# Autodesk Inventor assembly: MECANISMO DE COMPACTADO
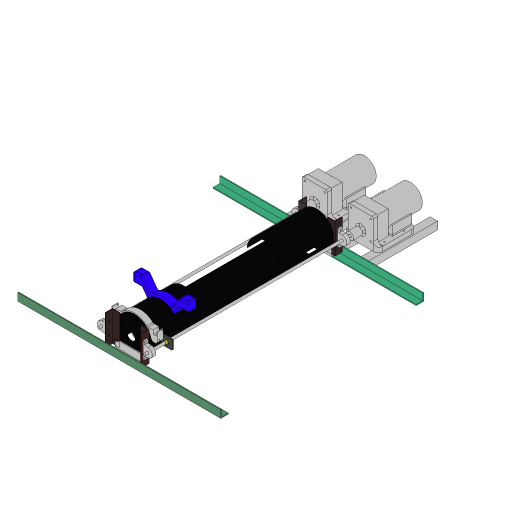
[picture p0: Inventor's stored thumbnail of the model, 512x512]
Saved by Autodesk Inventor 2024 (Build 280153000, 153)
## iProperties
Created: 2024-05-26
Part Number: MECANISMO DE COMPACTADO
Document SubType Name: Assembly
Designer: Jhuliams
Author: Jhuliams
## Documents named in this file (14)
- C:\Users\Jhuliams\Documents\GitHub\RECICLADOR_MODELO_3D\MECANISMO DE COMPACTADO\MECANISMO DE COMPACTADO.iam
- C:\Users\Jhuliams\Documents\GitHub\RECICLADOR_MODELO_3D\MECANISMO DE COMPACTADO\GUIA_DE_OBJETO.ipt
- C:\Users\Jhuliams\Documents\GitHub\RECICLADOR_MODELO_3D\MECANISMO DE COMPACTADO\TAPA QUE DESPLAZA CON TORNILLOS.ipt
- C:\Users\Jhuliams\Documents\GitHub\RECICLADOR_MODELO_3D\MECANISMO DE COMPACTADO\TUERCA DE HUSILLO.ipt
- C:\Users\Jhuliams\Documents\GitHub\RECICLADOR_MODELO_3D\MECANISMO DE COMPACTADO\TORNILLO DEPOTENCIA.ipt
- C:\Users\Jhuliams\Documents\GitHub\RECICLADOR_MODELO_3D\MECANISMO DE COMPACTADO\ACOPLE HELICOIDAL.ipt
- C:\Users\Jhuliams\Documents\GitHub\RECICLADOR_MODELO_3D\MECANISMO DE COMPACTADO\MOTOR DC.ipt
- C:\Users\Jhuliams\Documents\GitHub\RECICLADOR_MODELO_3D\MECANISMO DE COMPACTADO\RODAMIENTO DE TORNILLO.ipt
- C:\Users\Jhuliams\Documents\GitHub\RECICLADOR_MODELO_3D\MECANISMO DE COMPACTADO\SOPORTE DEL MOTOR.ipt
- C:\Users\Jhuliams\Documents\GitHub\RECICLADOR_MODELO_3D\MECANISMO DE COMPACTADO\SOPORTE LATERAL DE GUIA CILINDRICA.ipt
- C:\Users\Jhuliams\Documents\GitHub\RECICLADOR_MODELO_3D\MECANISMO DE COMPACTADO\PERFIL_SOPORTE DE CILINDRO.ipt
- C:\Users\Jhuliams\Documents\GitHub\RECICLADOR_MODELO_3D\MECANISMO DE COMPACTADO\PERFIL_SOPORTE DEL MOTOR.ipt
- C:\Users\Jhuliams\Documents\GitHub\RECICLADOR_MODELO_3D\MECANISMO DE COMPACTADO\SOPORTE DE SENSOR INFRARROJO.ipt
- C:\Users\Jhuliams\Documents\GitHub\RECICLADOR_MODELO_3D\MECANISMO DE COMPACTADO\SOPORTE FIN DE CARRERA.ipt
## Components (30 placed, 13 different names)
1. PERFIL_SOPORTE DE CILINDRO:1 — Mate:2, Flush:1, Mate:4, Flush:3, Mate:49
2. SOPORTE LATERAL DE GUIA CILINDRICA:5 — Mate:1, Mate:3, Mate:5, Flush:2, Mate:6, Mate:8
3. SOPORTE LATERAL DE GUIA CILINDRICA:6 — Mate:2, Mate:4, Mate:5, Flush:2, Mate:7
4. PERFIL_SOPORTE DE CILINDRO:3 — Mate:1, Flush:1, Mate:3, Flush:3, Flush:4, Flush:17
5. GUIA_DE_OBJETO:1 — Mate:6, Mate:7, Flush:4, Mate:8, Mate:9, Mate:10, Mate:34, Mate:35, Mate:65, Mate:66
6. TAPA QUE DESPLAZA CON TORNILLOS:1 — Mate:9, Mate:10, Mate:11, Mate:12, Mate:13, Mate:14, Mate:15
7. TUERCA DE HUSILLO:1 — Mate:12, Mate:13, Flush:5, Mate:15, Mate:16
8. TUERCA DE HUSILLO:2 — Mate:11, Mate:14, Flush:5, Mate:17
9. TORNILLO DEPOTENCIA:1 — Mate:16, Flush:6, Mate:30, Mate:33, Mate:36, Mate:37, Mate:39
10. TORNILLO DEPOTENCIA:2 — Mate:17, Flush:6, Mate:31, Mate:32, Mate:38, Mate:40
11. SOPORTE LATERAL DE GUIA CILINDRICA:7 — Mate:20, Mate:21, Mate:26, Flush:7, Flush:8, Mate:35, Flush:17
12. SOPORTE LATERAL DE GUIA CILINDRICA:8 — Mate:22, Mate:23, Mate:27, Flush:7, Flush:8
13. SOPORTE LATERAL DE GUIA CILINDRICA:9 — Mate:18, Mate:19, Mate:29, Flush:9, Flush:10, Mate:34
14. SOPORTE LATERAL DE GUIA CILINDRICA:10 — Mate:24, Mate:25, Mate:28, Flush:9, Flush:10
15. RODAMIENTO DE TORNILLO:1 — Mate:20, Mate:21, Mate:26, Mate:30, Mate:36
16. RODAMIENTO DE TORNILLO:2 — Mate:18, Mate:19, Mate:29, Mate:33
17. RODAMIENTO DE TORNILLO:3 — Mate:22, Mate:23, Mate:27, Mate:31
18. RODAMIENTO DE TORNILLO:4 — Mate:24, Mate:25, Mate:28, Mate:32
19. ACOPLE HELICOIDAL:1 — Mate:37, Mate:39, Mate:46, Mate:47
20. ACOPLE HELICOIDAL:2 — Mate:38, Mate:40, Mate:45, Mate:48
21. MOTOR DC:1 — Mate:41, Mate:42, Flush:12, Mate:46, Mate:47
22. MOTOR DC:2 — Mate:43, Mate:44, Flush:11, Mate:45, Mate:48
23. SOPORTE DEL MOTOR:1 — Mate:41, Mate:42, Flush:12, Mate:49, Flush:13, Mate:56, Mate:57, Mate:62, Mate:63, Mate:64
24. SOPORTE DEL MOTOR:2 — Mate:43, Mate:44, Flush:11, Flush:13, Mate:58, Mate:59, Mate:60, Mate:61
25. PERFIL_SOPORTE DEL MOTOR:2 — Mate:60, Mate:61, Flush:14
26. PERFIL_SOPORTE DEL MOTOR:4 — Mate:56, Mate:57, Flush:16, Mate:64
27. PERFIL_SOPORTE DEL MOTOR:5 — Mate:58, Mate:59, Flush:14, Flush:15
28. PERFIL_SOPORTE DEL MOTOR:6 — Mate:62, Mate:63, Flush:15, Flush:16
29. SOPORTE DE SENSOR INFRARROJO:1 — Mate:65
30. SOPORTE FIN DE CARRERA:1 — Mate:66
## Relationships (77: Mate 60, Flush 17)
- Mate:1: SOPORTE LATERAL DE GUIA CILINDRICA:5 ↔ PERFIL_SOPORTE DE CILINDRO:3
- Mate:2: PERFIL_SOPORTE DE CILINDRO:1 ↔ SOPORTE LATERAL DE GUIA CILINDRICA:6
- Flush:1: PERFIL_SOPORTE DE CILINDRO:1 ↔ PERFIL_SOPORTE DE CILINDRO:3
- Mate:3: SOPORTE LATERAL DE GUIA CILINDRICA:5 ↔ PERFIL_SOPORTE DE CILINDRO:3
- Mate:4: PERFIL_SOPORTE DE CILINDRO:1 ↔ SOPORTE LATERAL DE GUIA CILINDRICA:6
- Mate:5 (626 mm): SOPORTE LATERAL DE GUIA CILINDRICA:5 ↔ SOPORTE LATERAL DE GUIA CILINDRICA:6
- Flush:2: SOPORTE LATERAL DE GUIA CILINDRICA:5 ↔ SOPORTE LATERAL DE GUIA CILINDRICA:6
- Flush:3: PERFIL_SOPORTE DE CILINDRO:1 ↔ PERFIL_SOPORTE DE CILINDRO:3
- Mate:6: SOPORTE LATERAL DE GUIA CILINDRICA:5 ↔ GUIA_DE_OBJETO:1
- Mate:7: SOPORTE LATERAL DE GUIA CILINDRICA:6 ↔ GUIA_DE_OBJETO:1
- Flush:4 (-51.5 mm): PERFIL_SOPORTE DE CILINDRO:3 ↔ GUIA_DE_OBJETO:1
- Mate:8 (-50 mm): SOPORTE LATERAL DE GUIA CILINDRICA:5 ↔ GUIA_DE_OBJETO:1
- Mate:9: GUIA_DE_OBJETO:1 ↔ TAPA QUE DESPLAZA CON TORNILLOS:1
- Mate:10 (1 mm): GUIA_DE_OBJETO:1 ↔ TAPA QUE DESPLAZA CON TORNILLOS:1
- Mate:11: TAPA QUE DESPLAZA CON TORNILLOS:1 ↔ TUERCA DE HUSILLO:2
- Mate:12: TAPA QUE DESPLAZA CON TORNILLOS:1 ↔ TUERCA DE HUSILLO:1
- Mate:13: TAPA QUE DESPLAZA CON TORNILLOS:1 ↔ TUERCA DE HUSILLO:1
- Mate:14: TAPA QUE DESPLAZA CON TORNILLOS:1 ↔ TUERCA DE HUSILLO:2
- Flush:5: TUERCA DE HUSILLO:1 ↔ TUERCA DE HUSILLO:2
- Mate:15: TAPA QUE DESPLAZA CON TORNILLOS:1 ↔ TUERCA DE HUSILLO:1
- Mate:16: TUERCA DE HUSILLO:1 ↔ TORNILLO DEPOTENCIA:1
- Mate:17: TUERCA DE HUSILLO:2 ↔ TORNILLO DEPOTENCIA:2
- Flush:6: TORNILLO DEPOTENCIA:1 ↔ TORNILLO DEPOTENCIA:2
- Mate:18: SOPORTE LATERAL DE GUIA CILINDRICA:9 ↔ RODAMIENTO DE TORNILLO:2
- Mate:19: SOPORTE LATERAL DE GUIA CILINDRICA:9 ↔ RODAMIENTO DE TORNILLO:2
- Mate:20: SOPORTE LATERAL DE GUIA CILINDRICA:7 ↔ RODAMIENTO DE TORNILLO:1
- Mate:21: SOPORTE LATERAL DE GUIA CILINDRICA:7 ↔ RODAMIENTO DE TORNILLO:1
- Mate:22: SOPORTE LATERAL DE GUIA CILINDRICA:8 ↔ RODAMIENTO DE TORNILLO:3
- Mate:23: SOPORTE LATERAL DE GUIA CILINDRICA:8 ↔ RODAMIENTO DE TORNILLO:3
- Mate:24: SOPORTE LATERAL DE GUIA CILINDRICA:10 ↔ RODAMIENTO DE TORNILLO:4
- Mate:25: SOPORTE LATERAL DE GUIA CILINDRICA:10 ↔ RODAMIENTO DE TORNILLO:4
- Mate:26: SOPORTE LATERAL DE GUIA CILINDRICA:7 ↔ RODAMIENTO DE TORNILLO:1
- Mate:27: SOPORTE LATERAL DE GUIA CILINDRICA:8 ↔ RODAMIENTO DE TORNILLO:3
- Mate:28: SOPORTE LATERAL DE GUIA CILINDRICA:10 ↔ RODAMIENTO DE TORNILLO:4
- Mate:29: SOPORTE LATERAL DE GUIA CILINDRICA:9 ↔ RODAMIENTO DE TORNILLO:2
- Flush:7: SOPORTE LATERAL DE GUIA CILINDRICA:7 ↔ SOPORTE LATERAL DE GUIA CILINDRICA:8
- Flush:8: SOPORTE LATERAL DE GUIA CILINDRICA:7 ↔ SOPORTE LATERAL DE GUIA CILINDRICA:8
- Flush:9: SOPORTE LATERAL DE GUIA CILINDRICA:9 ↔ SOPORTE LATERAL DE GUIA CILINDRICA:10
- Flush:10: SOPORTE LATERAL DE GUIA CILINDRICA:9 ↔ SOPORTE LATERAL DE GUIA CILINDRICA:10
- Mate:30: TORNILLO DEPOTENCIA:1 ↔ RODAMIENTO DE TORNILLO:1
- Mate:31: TORNILLO DEPOTENCIA:2 ↔ RODAMIENTO DE TORNILLO:3
- Mate:32: TORNILLO DEPOTENCIA:2 ↔ RODAMIENTO DE TORNILLO:4
- Mate:33: TORNILLO DEPOTENCIA:1 ↔ RODAMIENTO DE TORNILLO:2
- Mate:34: GUIA_DE_OBJETO:1 ↔ SOPORTE LATERAL DE GUIA CILINDRICA:9
- Mate:35: GUIA_DE_OBJETO:1 ↔ SOPORTE LATERAL DE GUIA CILINDRICA:7
- Mate:36 (-10 mm): TORNILLO DEPOTENCIA:1 ↔ RODAMIENTO DE TORNILLO:1
- Mate:37: TORNILLO DEPOTENCIA:1 ↔ ACOPLE HELICOIDAL:1
- Mate:38: TORNILLO DEPOTENCIA:2 ↔ ACOPLE HELICOIDAL:2
- Mate:39 (-10 mm): TORNILLO DEPOTENCIA:1 ↔ ACOPLE HELICOIDAL:1
- Mate:40 (-10 mm): TORNILLO DEPOTENCIA:2 ↔ ACOPLE HELICOIDAL:2
- Mate:41: MOTOR DC:1 ↔ SOPORTE DEL MOTOR:1
- Mate:42: MOTOR DC:1 ↔ SOPORTE DEL MOTOR:1
- Mate:43: MOTOR DC:2 ↔ SOPORTE DEL MOTOR:2
- Mate:44: MOTOR DC:2 ↔ SOPORTE DEL MOTOR:2
- Flush:11 (2.5 mm): MOTOR DC:2 ↔ SOPORTE DEL MOTOR:2
- Flush:12 (2.5 mm): MOTOR DC:1 ↔ SOPORTE DEL MOTOR:1
- Mate:45: ACOPLE HELICOIDAL:2 ↔ MOTOR DC:2
- Mate:46: ACOPLE HELICOIDAL:1 ↔ MOTOR DC:1
- Mate:47 (-10 mm): ACOPLE HELICOIDAL:1 ↔ MOTOR DC:1
- Mate:48 (-10 mm): ACOPLE HELICOIDAL:2 ↔ MOTOR DC:2
- Mate:49 (15 mm): PERFIL_SOPORTE DE CILINDRO:1 ↔ SOPORTE DEL MOTOR:1
- Flush:13: SOPORTE DEL MOTOR:1 ↔ SOPORTE DEL MOTOR:2
- Mate:56: SOPORTE DEL MOTOR:1 ↔ PERFIL_SOPORTE DEL MOTOR:4
- Mate:57: SOPORTE DEL MOTOR:1 ↔ PERFIL_SOPORTE DEL MOTOR:4
- Mate:58: SOPORTE DEL MOTOR:2 ↔ PERFIL_SOPORTE DEL MOTOR:5
- Mate:59: SOPORTE DEL MOTOR:2 ↔ PERFIL_SOPORTE DEL MOTOR:5
- Mate:60: SOPORTE DEL MOTOR:2 ↔ PERFIL_SOPORTE DEL MOTOR:2
- Mate:61: SOPORTE DEL MOTOR:2 ↔ PERFIL_SOPORTE DEL MOTOR:2
- Mate:62: SOPORTE DEL MOTOR:1 ↔ PERFIL_SOPORTE DEL MOTOR:6
- Mate:63: SOPORTE DEL MOTOR:1 ↔ PERFIL_SOPORTE DEL MOTOR:6
- Flush:14: PERFIL_SOPORTE DEL MOTOR:2 ↔ PERFIL_SOPORTE DEL MOTOR:5
- Flush:15: PERFIL_SOPORTE DEL MOTOR:5 ↔ PERFIL_SOPORTE DEL MOTOR:6
- Flush:16: PERFIL_SOPORTE DEL MOTOR:4 ↔ PERFIL_SOPORTE DEL MOTOR:6
- Mate:64: SOPORTE DEL MOTOR:1 ↔ PERFIL_SOPORTE DEL MOTOR:4
- Flush:17 (270 mm): PERFIL_SOPORTE DE CILINDRO:3 ↔ SOPORTE LATERAL DE GUIA CILINDRICA:7
- Mate:65: GUIA_DE_OBJETO:1 ↔ SOPORTE DE SENSOR INFRARROJO:1
- Mate:66: GUIA_DE_OBJETO:1 ↔ SOPORTE FIN DE CARRERA:1
